# Autodesk Inventor assembly: subassembly_auger_case
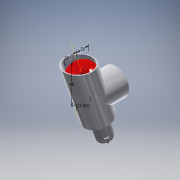
[picture p0: Inventor's stored thumbnail of the model, 180x180]
Saved by Autodesk Inventor 2019 (Build 230136000, 136)
## iProperties
Created: 2019-01-23
Part Number: subassembly_auger_case
Document SubType Name: Assembly
Designer: jmc
Author: jmc
## Documents named in this file (4)
- C:\Users\l0086\Desktop\Models\CatFeeder\version4 (auger)\subassembly_auger_case.iam
- C:\Users\l0086\Desktop\Models\3party\DCMotor\12dcmotorDC Motor 12V.iam
- C:\Users\l0086\Desktop\Models\CatFeeder\Auger\auger.ipt
- C:\Users\l0086\Desktop\Models\CatFeeder\Auger\screw.ipt
## Components (3 placed, 3 different names)
1. 12dcmotorDC Motor 12V:1 [sub-assembly] — Rotational:2
2. auger:1 — Rotational:1
3. screw:1 — Rotational:1, Rotational:2
## Relationships (2: RevoluteJoint 2)
- Rotational:1 [RevoluteJoint]: auger:1 ↔ screw:1
- Rotational:2 [RevoluteJoint]: 12dcmotorDC Motor 12V:1 ↔ screw:1
